# Autodesk Inventor assembly: Manubrio_ruta
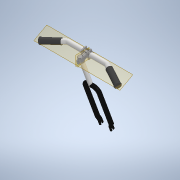
[picture p0: Inventor's stored thumbnail of the model, 180x180]
Saved by Autodesk Inventor 2021 (Build 250183000, 183)
## iProperties
Created: 2021-04-24
Part Number: Manubrio_ruta
Document SubType Name: Assembly
Designer: maaro
Author: maaro
## Documents named in this file (10)
- C:\Git\Proyecto_APM\02 Inventor\bicicleta_ruta\Manubrio\Manubrio_ruta.iam
- C:\Git\Proyecto_APM\02 Inventor\bicicleta_ruta\Manubrio\Mango Der.ipt
- C:\Git\Proyecto_APM\02 Inventor\bicicleta_ruta\Manubrio\Mango Izq.ipt
- C:\Git\Proyecto_APM\02 Inventor\bicicleta_ruta\Manubrio\Copa Tenedor.ipt
- C:\Git\Proyecto_APM\02 Inventor\bicicleta_ruta\Manubrio\Tubo Tenedor Izq.ipt
- C:\Git\Proyecto_APM\02 Inventor\bicicleta_ruta\Manubrio\Tubo Tenedor Der.ipt
- C:\Git\Proyecto_APM\02 Inventor\bicicleta_ruta\Manubrio\Tubo Tenedor Central.ipt
- C:\Git\Proyecto_APM\02 Inventor\bicicleta_ruta\Manubrio\Potencia Tras.ipt
- C:\Git\Proyecto_APM\02 Inventor\bicicleta_ruta\Manubrio\Potencia Del.ipt
- C:\Git\Proyecto_APM\02 Inventor\bicicleta_ruta\caña bici ruta.ipt
## Components (9 placed, 9 different names)
1. Mango Der:1 — Mate:2, Mate:4
2. Mango Izq:1 — Mate:3, Mate:5
3. Copa Tenedor:1
4. Tubo Tenedor Izq:1
5. Tubo Tenedor Der:1
6. Tubo Tenedor Central:1
7. Potencia Tras:1 — Mate:1
8. Potencia Del:1 — Mate:6
9. caña bici ruta:1 — Mate:1, Mate:2, Mate:3, Mate:4, Mate:5, Mate:6
## Relationships (6: Mate 6)
- Mate:1: Potencia Tras:1 ↔ caña bici ruta:1
- Mate:2: Mango Der:1 ↔ caña bici ruta:1
- Mate:3: Mango Izq:1 ↔ caña bici ruta:1
- Mate:4: Mango Der:1 ↔ caña bici ruta:1
- Mate:5: Mango Izq:1 ↔ caña bici ruta:1
- Mate:6: Potencia Del:1 ↔ caña bici ruta:1
